# Autodesk Inventor assembly: Tension_Bearings
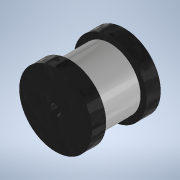
[picture p0: Inventor's stored thumbnail of the model, 180x180]
Saved by Autodesk Inventor 2022 (Build 260153000, 153)
## iProperties
Created: 2022-03-16
Part Number: Tension_Bearings
Document SubType Name: Assembly
Designer: Mlees
Author: Mlees
## Documents named in this file (4)
- C:\Users\Mlees\Desktop\504Engineering\Stepper-Servo_Based_Robotic_Arm\Designs\Version_8\Created_Parts\Tension_Bearings.iam
- C:\Users\Mlees\Desktop\504Engineering\Stepper-Servo_Based_Robotic_Arm\Designs\Version_8\Created_Parts\Belt_Bearing_Holder_p2.ipt
- C:\Users\Mlees\Desktop\504Engineering\Stepper-Servo_Based_Robotic_Arm\Designs\Version_8\Created_Parts\Belt_Bearing_Holder.ipt
- C:\Users\Mlees\Desktop\504Engineering\Stepper-Servo_Based_Robotic_Arm\Designs\Version_8\Created_Parts\Belt_Tension_Bearing.ipt
## Components (4 placed, 3 different names)
1. Belt_Bearing_Holder_p2:1 — Mate:3
2. Belt_Bearing_Holder:1 — Mate:1, Mate:3
3. Belt_Tension_Bearing:1 — Mate:2
4. Belt_Tension_Bearing:2 — Mate:1, Mate:2
## Relationships (3: Mate 3)
- Mate:1: Belt_Bearing_Holder:1 ↔ Belt_Tension_Bearing:2
- Mate:2: Belt_Tension_Bearing:1 ↔ Belt_Tension_Bearing:2
- Mate:3: Belt_Bearing_Holder_p2:1 ↔ Belt_Bearing_Holder:1
